# Autodesk Inventor assembly: Should Be Ball Suck
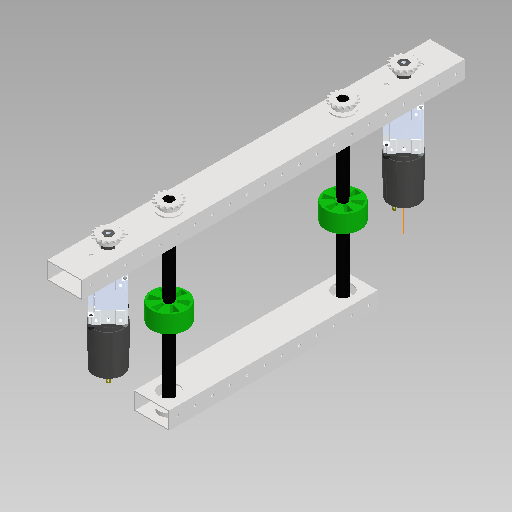
[picture p0: Inventor's stored thumbnail of the model, 512x512]
Saved by Autodesk Inventor 2021 (Build 250183000, 183)
## iProperties
Created: 2021-02-10
Part Number: Should Be Ball Suck
Document SubType Name: Assembly
Designer: aidan
Author: aidan
## Documents named in this file (9)
- C:\Users\Merkileg\Documents\t3-cad\CAD\2021 Specific Parts\Should Be Ball Suck.iam
- C:\Users\Merkileg\Documents\t3-cad\CAD\2021 Specific Parts\VerseFrame 12in for BS.ipt
- C:\Users\Merkileg\Documents\t3-cad\CAD\Generic and Stock\VersaPlanetary v2 Two Stage Shrinkwrap.ipt
- C:\Users\Merkileg\Documents\t3-cad\CAD\Generic and Stock\775 Pro.ipt
- C:\Users\Merkileg\Documents\t3-cad\CAD\2021 Specific Parts\VerseFrame 22in for Ball Suck.ipt
- C:\Users\Merkileg\Documents\t3-cad\CAD\Generic and Stock\16T 22 Sprocket.ipt
- C:\Users\Merkileg\Documents\t3-cad\CAD\Bearing for THUNDER.ipt
- C:\Users\Merkileg\Documents\t3-cad\CAD\Tony's CAD\Compliance wheel.ipt
- C:\Users\Merkileg\Documents\t3-cad\CAD\10.75in THUNDERSHAFT.ipt
## Components (18 placed, 8 different names)
1. VerseFrame 12in for BS:2 — Flush:6, Mate:11, Mate:12, Mate:25, Mate:27
2. VersaPlanetary v2 Two Stage Shrinkwrap:1 — Flush:4, Mate:2, Mate:6, Mate:8, Mate:16, Mate:18, Mate:19, Flush:8
3. VersaPlanetary v2 Two Stage Shrinkwrap:2 — Flush:4, Mate:3, Mate:15, Mate:17, Mate:20, Mate:21
4. 775 Pro:1 — Flush:5, Mate:4, Mate:6
5. 775 Pro:2 — Flush:5, Mate:5, Mate:10
6. VerseFrame 22in for Ball Suck:1 — Mate:8, Mate:9, Mate:10, Flush:6, Mate:11, Mate:12, Mate:15, Mate:16, Mate:17, Mate:24, Mate:26, Mate:39
7. 16T 22 Sprocket:1 — Mate:18, Mate:19, Flush:7, Flush:8
8. 16T 22 Sprocket:2 — Mate:20, Mate:21, Flush:7
9. Bearing for THUNDER:1 — Mate:22, Flush:9, Mate:28, Mate:30, Mate:38
10. Bearing for THUNDER:2 — Mate:23, Flush:9, Mate:26, Mate:29, Mate:31
11. Bearing for THUNDER:3 — Mate:22, Mate:25, Flush:10, Mate:27
12. Bearing for THUNDER:4 — Mate:23, Mate:24, Flush:10
13. 16T 22 Sprocket:3 — Mate:34, Mate:36, Flush:19, Flush:20, Mate:38
14. 16T 22 Sprocket:4 — Mate:35, Mate:37, Flush:19
15. 10.75in THUNDERSHAFT:1 — Mate:28, Flush:17, Mate:30, Mate:32, Mate:34, Mate:36, Flush:20
16. 10.75in THUNDERSHAFT:2 — Mate:29, Flush:17, Mate:31, Mate:33, Mate:35, Mate:37
17. Compliance wheel:1 — Flush:18, Mate:32, Mate:39
18. Compliance wheel:2 — Flush:18, Mate:33
## Relationships (46: Mate 35, Flush 11)
- Flush:4: VersaPlanetary v2 Two Stage Shrinkwrap:1 ↔ VersaPlanetary v2 Two Stage Shrinkwrap:2
- Flush:5: 775 Pro:1 ↔ 775 Pro:2
- Mate:2: VersaPlanetary v2 Two Stage Shrinkwrap:1
- Mate:3: VersaPlanetary v2 Two Stage Shrinkwrap:2
- Mate:4: 775 Pro:1
- Mate:5: 775 Pro:2
- Mate:6: VersaPlanetary v2 Two Stage Shrinkwrap:1 ↔ 775 Pro:1
- Mate:8: VersaPlanetary v2 Two Stage Shrinkwrap:1 ↔ VerseFrame 22in for Ball Suck:1
- Mate:9: VerseFrame 22in for Ball Suck:1
- Mate:10: 775 Pro:2 ↔ VerseFrame 22in for Ball Suck:1
- Flush:6: VerseFrame 12in for BS:2 ↔ VerseFrame 22in for Ball Suck:1
- Mate:11 (203.2 mm): VerseFrame 12in for BS:2 ↔ VerseFrame 22in for Ball Suck:1
- Mate:12: VerseFrame 12in for BS:2 ↔ VerseFrame 22in for Ball Suck:1
- Mate:15: VersaPlanetary v2 Two Stage Shrinkwrap:2 ↔ VerseFrame 22in for Ball Suck:1
- Mate:16: VersaPlanetary v2 Two Stage Shrinkwrap:1 ↔ VerseFrame 22in for Ball Suck:1
- Mate:17: VersaPlanetary v2 Two Stage Shrinkwrap:2 ↔ VerseFrame 22in for Ball Suck:1
- Mate:18: VersaPlanetary v2 Two Stage Shrinkwrap:1 ↔ 16T 22 Sprocket:1
- Mate:19: VersaPlanetary v2 Two Stage Shrinkwrap:1 ↔ 16T 22 Sprocket:1
- Mate:20: VersaPlanetary v2 Two Stage Shrinkwrap:2 ↔ 16T 22 Sprocket:2
- Mate:21: VersaPlanetary v2 Two Stage Shrinkwrap:2 ↔ 16T 22 Sprocket:2
- Flush:7: 16T 22 Sprocket:1 ↔ 16T 22 Sprocket:2
- Flush:8: VersaPlanetary v2 Two Stage Shrinkwrap:1 ↔ 16T 22 Sprocket:1
- Mate:22: Bearing for THUNDER:1 ↔ Bearing for THUNDER:3
- Mate:23: Bearing for THUNDER:2 ↔ Bearing for THUNDER:4
- Mate:24: VerseFrame 22in for Ball Suck:1 ↔ Bearing for THUNDER:4
- Mate:25: VerseFrame 12in for BS:2 ↔ Bearing for THUNDER:3
- Flush:9: Bearing for THUNDER:1 ↔ Bearing for THUNDER:2
- Mate:26: VerseFrame 22in for Ball Suck:1 ↔ Bearing for THUNDER:2
- Flush:10: Bearing for THUNDER:3 ↔ Bearing for THUNDER:4
- Mate:27: VerseFrame 12in for BS:2 ↔ Bearing for THUNDER:3
- Mate:28: Bearing for THUNDER:1 ↔ 10.75in THUNDERSHAFT:1
- Mate:29: Bearing for THUNDER:2 ↔ 10.75in THUNDERSHAFT:2
- Flush:17: 10.75in THUNDERSHAFT:1 ↔ 10.75in THUNDERSHAFT:2
- Mate:30: Bearing for THUNDER:1 ↔ 10.75in THUNDERSHAFT:1
- Mate:31: Bearing for THUNDER:2 ↔ 10.75in THUNDERSHAFT:2
- Flush:18: Compliance wheel:1 ↔ Compliance wheel:2
- Mate:32: 10.75in THUNDERSHAFT:1 ↔ Compliance wheel:1
- Mate:33: 10.75in THUNDERSHAFT:2 ↔ Compliance wheel:2
- Mate:34: 16T 22 Sprocket:3 ↔ 10.75in THUNDERSHAFT:1
- Mate:35: 16T 22 Sprocket:4 ↔ 10.75in THUNDERSHAFT:2
- Mate:36 (0.0127 mm): 16T 22 Sprocket:3 ↔ 10.75in THUNDERSHAFT:1
- Mate:37 (0.0127 mm): 16T 22 Sprocket:4 ↔ 10.75in THUNDERSHAFT:2
- Flush:19: 16T 22 Sprocket:3 ↔ 16T 22 Sprocket:4
- Flush:20: 16T 22 Sprocket:3 ↔ 10.75in THUNDERSHAFT:1
- Mate:38 (3.175 mm): Bearing for THUNDER:1 ↔ 16T 22 Sprocket:3
- Mate:39 (88.9 mm): VerseFrame 22in for Ball Suck:1 ↔ Compliance wheel:1
